# Autodesk Inventor assembly: x-IMU 2 Housing
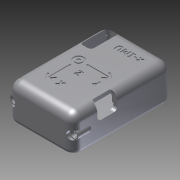
[picture p0: Inventor's stored thumbnail of the model, 180x180]
Saved by Autodesk Inventor 2011 (Build 150239000, 239)
## iProperties
Created: 2011-08-18
Part Number: x-IMU 2 Housing
Document SubType Name: Assembly
Designer: Jacky
Author: Jacky
## Documents named in this file (3)
- C:\MyFiles\x-io\Products\x-IMU\x-IMU Mechanical\x-IMU v1.4 Housing\x-IMU 1.4 Housing.iam
- C:\MyFiles\x-io\Products\x-IMU\x-IMU Mechanical\x-IMU v1.4 Housing\x-IMU 1.4 Housing - MainHollowedMezzanine Mk2.ipt
- C:\MyFiles\x-io\Products\x-IMU\x-IMU Mechanical\x-IMU v1.4 Housing\x-IMU 1.4 Housing - Lid Mk2.ipt
## Components (2 placed, 2 different names)
1. x-IMU 1.4 Housing - MainHollowedMezzanine Mk2:1 — Insert:1, Insert:2
2. x-IMU 1.4 Housing - Lid Mk2:1 — Insert:1, Insert:2
## Relationships (2: Insert 2)
- Insert:1: x-IMU 1.4 Housing - MainHollowedMezzanine Mk2:1 ↔ x-IMU 1.4 Housing - Lid Mk2:1
- Insert:2: x-IMU 1.4 Housing - MainHollowedMezzanine Mk2:1 ↔ x-IMU 1.4 Housing - Lid Mk2:1
